# Autodesk Inventor assembly: FanAssembly
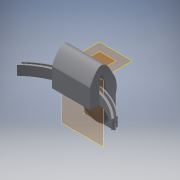
[picture p0: Inventor's stored thumbnail of the model, 180x180]
Saved by Autodesk Inventor 2016 (Build 200138000, 138)
## iProperties
Created: 2016-08-18
Part Number: FanAssembly
Document SubType Name: Assembly
Designer: yash
Author: yash
## Documents named in this file (5)
- C:\Users\yash\Documents\GitHub\ClipFanHat\FanAssembly.iam
- C:\Users\yash\Documents\GitHub\ClipFanHat\FanLip.ipt
- C:\Users\yash\Documents\GitHub\ClipFanHat\Vent.ipt
- C:\Users\yash\Documents\GitHub\ClipFanHat\Clip.ipt
- C:\Users\yash\Documents\GitHub\ClipFanHat\ClipBottom.ipt
## Components (4 placed, 4 different names)
1. FanLip:1 — Insert:1
2. Vent:1 — Insert:1, Mate:1, Mate:2, Mate:3
3. Clip:1 — Flush:1, Flush:2, Flush:3, Flush:4, Mate:4
4. ClipBottom:1 — Mate:1, Mate:2, Mate:3, Flush:1, Flush:2, Flush:3, Flush:4, Mate:4
## Relationships (9: Mate 4, Flush 4, Insert 1)
- Insert:1: FanLip:1 ↔ Vent:1
- Mate:1: Vent:1 ↔ ClipBottom:1
- Mate:2: Vent:1 ↔ ClipBottom:1
- Mate:3: Vent:1 ↔ ClipBottom:1
- Flush:1: Clip:1 ↔ ClipBottom:1
- Flush:2: Clip:1 ↔ ClipBottom:1
- Flush:3: Clip:1 ↔ ClipBottom:1
- Flush:4: Clip:1 ↔ ClipBottom:1
- Mate:4 (3.175 mm): Clip:1 ↔ ClipBottom:1
